# Autodesk Inventor assembly: Assembled box
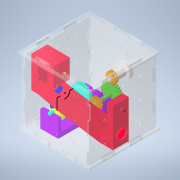
[picture p0: Inventor's stored thumbnail of the model, 180x180]
Saved by Autodesk Inventor 2021 (Build 250183000, 183)
## iProperties
Created: 2020-02-27
Part Number: Assembled box
Document SubType Name: Assembly
Designer: jstr255
Author: jstr255
## Documents named in this file (19)
- C:\Users\Jawal\Documents\UNI\PART III\Semester 1\MECHENG 334\Project A\CAD Files\Assemblies\Assembly `\Assembled_box.iam
- C:\Users\Jawal\Documents\UNI\PART III\Semester 1\MECHENG 334\Project A\CAD Files\Main\Main_Assembly_export\Box base.ipt
- C:\Users\Jawal\Documents\UNI\PART III\Semester 1\MECHENG 334\Project A\CAD Files\Main\Main_Assembly_export\Box side 1.ipt
- C:\Users\Jawal\Documents\UNI\PART III\Semester 1\MECHENG 334\Project A\CAD Files\Main\Main_Assembly_export\Box side 2.ipt
- C:\Users\Jawal\Documents\UNI\PART III\Semester 1\MECHENG 334\Project A\CAD Files\Main\Main_Assembly_export\Box side 3.ipt
- C:\Users\Jawal\Documents\UNI\PART III\Semester 1\MECHENG 334\Project A\CAD Files\Main\Main_Assembly_export\Box side 4.ipt
- C:\Users\Jawal\Documents\UNI\PART III\Semester 1\MECHENG 334\Project A\CAD Files\Main\Main_Assembly_export\Box top.ipt
- C:\Users\Jawal\Documents\UNI\PART III\Semester 1\MECHENG 334\Project A\CAD Files\NA Assembly\Main_Assembly_export\Driveshaft coupling end.ipt
- C:\Users\Jawal\Documents\UNI\PART III\Semester 1\MECHENG 334\Project A\CAD Files\NA Assembly\Main_Assembly_export\Input Connection.ipt
- C:\Users\Jawal\Documents\UNI\PART III\Semester 1\MECHENG 334\Project A\CAD Files\Main\Main_Assembly_export\Final Spur Gear Large.ipt
- C:\Users\Jawal\Documents\UNI\PART III\Semester 1\MECHENG 334\Project A\CAD Files\Main\Main_Assembly_export\Spur Gear12.ipt
- C:\Users\Jawal\Documents\UNI\PART III\Semester 1\MECHENG 334\Project A\CAD Files\NA Assembly\Main_Assembly_export\Extra Shaft.ipt
- C:\Users\Jawal\Documents\UNI\PART III\Semester 1\MECHENG 334\Project A\CAD Files\Assemblies\Assembly `\top_part.ipt
- C:\Users\Jawal\Documents\UNI\PART III\Semester 1\MECHENG 334\Project A\CAD Files\Assemblies\Assembly `\Block.ipt
- C:\Users\Jawal\Documents\UNI\PART III\Semester 1\MECHENG 334\Project A\CAD Files\Assemblies\Assembly `\Cam_4.ipt
- C:\Users\Jawal\Documents\UNI\PART III\Semester 1\MECHENG 334\Project A\CAD Files\Assemblies\Assembly `\bottom_part.ipt
- C:\Users\Jawal\Documents\UNI\PART III\Semester 1\MECHENG 334\Project A\CAD Files\Assemblies\Assembly `\shaft_support.ipt
- C:\Users\Jawal\Documents\UNI\PART III\Semester 1\MECHENG 334\Project A\CAD Files\Assemblies\Assembly `\support_2.ipt
- C:\Users\Jawal\Documents\UNI\PART III\Semester 1\MECHENG 334\Project A\CAD Files\Assemblies\Assembly `\Spur_Gear12.ipt
## Components (19 placed, 17 different names)
1. Box base:1 — Mate:1, Mate:2, Mate:3, Mate:4, Mate:5, Mate:6, Mate:7, Mate:8, Mate:9, Mate:10, Flush:4, Mate:30, Mate:33, Rigid:21, Rigid:22
2. Box side 1:1 — Mate:1, Mate:2, Mate:3, Flush:1, Mate:14, Rotational:1
3. Box side 2:1 — Mate:4, Mate:5, Mate:6, Mate:13, Rigid:17
4. Box side 3:1 — Mate:7, Mate:8, Mate:9, Mate:11
5. Box side 4:1 — Mate:10, Mate:11, Flush:1, Mate:12, Flush:2, Mate:26, Flush:14, Flush:15, Rigid:9, Flush:18
6. Box top:1 — Mate:12, Mate:13, Mate:14
7. Driveshaft coupling end:2 — Rotational:1, Mate:15, Mate:16, Mate:17, Angle:1
8. Input Connection:1 — Mate:15, Mate:16, Mate:17, Rigid:18
9. Spur Gear2:1 — Mate:24, Flush:11, Rotation:2, Mate:26, Mate:30, Rigid:19
10. Spur Gear1:1 — Mate:24, Flush:11, Rotation:2, Rigid:18
11. Spur Gear1:2 — Rigid:19, Flush:20, Mate:32, Rotation:3
12. Extra Shaft:1
13. top_part:1 — Rigid:9, Mate:34, Mate:35
14. Block:1 — Mate:34, Mate:35, Transitional:1
15. Cam_4:1 — Rigid:20, Transitional:1
16. bottom_part:1 — Rigid:17
17. Spur Gear2:2 — Flush:20, Mate:32, Mate:33, Rotation:3, Rigid:20, Mate:36
18. shaft_support:1 — Rigid:21
19. support_2:1 — Rigid:22
## Relationships (45: Mate 25, Flush 8, WeldJoint 7, RelateRotation 2, RevoluteJoint 1, Angle 1, Transitional 1)
- Mate:1: Box base:1 ↔ Box side 1:1
- Mate:2: Box base:1 ↔ Box side 1:1
- Mate:3: Box base:1 ↔ Box side 1:1
- Mate:4: Box base:1 ↔ Box side 2:1
- Mate:5: Box base:1 ↔ Box side 2:1
- Mate:6: Box base:1 ↔ Box side 2:1
- Mate:7: Box base:1 ↔ Box side 3:1
- Mate:8: Box base:1 ↔ Box side 3:1
- Mate:9: Box base:1 ↔ Box side 3:1
- Mate:10: Box base:1 ↔ Box side 4:1
- Mate:11: Box side 3:1 ↔ Box side 4:1
- Flush:1: Box side 1:1 ↔ Box side 4:1
- Mate:12: Box side 4:1 ↔ Box top:1
- Mate:13: Box side 2:1 ↔ Box top:1
- Mate:14: Box side 1:1 ↔ Box top:1
- Rotational:1 [RevoluteJoint]: Box side 1:1 ↔ Driveshaft coupling end:2
- Mate:15: Driveshaft coupling end:2 ↔ Input Connection:1
- Mate:16: Driveshaft coupling end:2 ↔ Input Connection:1
- Mate:17: Driveshaft coupling end:2 ↔ Input Connection:1
- Flush:2 (50 mm): Box side 4:1
- Flush:4 (50 mm): Box base:1
- Mate:24 (22.5 mm): Spur Gear2:1 ↔ Spur Gear1:1
- Flush:11: Spur Gear2:1 ↔ Spur Gear1:1
- Rotation:2 [RelateRotation] (0.5 ul): Spur Gear2:1 ↔ Spur Gear1:1
- Mate:26 (50 mm): Box side 4:1 ↔ Spur Gear2:1
- Mate:30 (27.5 mm): Box base:1 ↔ Spur Gear2:1
- Flush:14 (27.503 mm): Box side 4:1
- Angle:1 (0 deg): Driveshaft coupling end:2
- Flush:15 (27.503 mm): Box side 4:1
- Rigid:9 [WeldJoint]: Box side 4:1 ↔ top_part:1
- Flush:18 (27.503 mm): Box side 4:1
- Rigid:17 [WeldJoint]: Box side 2:1 ↔ bottom_part:1
- Rigid:18 [WeldJoint]: Input Connection:1 ↔ Spur Gear1:1
- Rigid:19 [WeldJoint]: Spur Gear2:1 ↔ Spur Gear1:2
- Flush:20: Spur Gear1:2 ↔ Spur Gear2:2
- Mate:32 (22.5 mm): Spur Gear1:2 ↔ Spur Gear2:2
- Mate:33 (27.147 mm): Box base:1 ↔ Spur Gear2:2
- Rotation:3 [RelateRotation] (2 ul): Spur Gear1:2 ↔ Spur Gear2:2
- Rigid:20 [WeldJoint] (6 mm): Cam_4:1 ↔ Spur Gear2:2
- Mate:34 (0.5 mm): top_part:1 ↔ Block:1
- Mate:35 (0.5 mm): top_part:1 ↔ Block:1
- Rigid:21 [WeldJoint]: Box base:1 ↔ shaft_support:1
- Rigid:22 [WeldJoint]: Box base:1 ↔ support_2:1
- Mate:36 (66.038 mm): Spur Gear2:2
- Transitional:1: Block:1 ↔ Cam_4:1
